# Autodesk Inventor assembly: Plac_Log
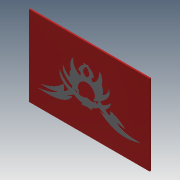
[picture p0: Inventor's stored thumbnail of the model, 180x180]
Saved by Autodesk Inventor 2019 (Build 230136000, 136)
## iProperties
Created: 2019-08-01
Part Number: Plac_Log
Document SubType Name: Assembly
Designer: giacomo
Author: giacomo
## Documents named in this file (3)
- D:\Hobby\Inventor\Case 3Dprinted\Placchetta\Plac_Log.iam
- D:\Hobby\Inventor\Case 3Dprinted\Placchetta\Logo.ipt
- D:\Hobby\Inventor\Case 3Dprinted\Placchetta\Placchetta.ipt
## Components (2 placed, 2 different names)
1. Logo:2 — Mate:1
2. Placchetta:1 — Mate:1
## Relationships (1: Mate 1)
- Mate:1: Logo:2 ↔ Placchetta:1
